# Autodesk Inventor assembly: Assembly_Cube_Lens_holder_v3
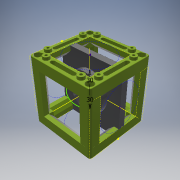
[picture p0: Inventor's stored thumbnail of the model, 180x180]
Saved by Autodesk Inventor 2019 (Build 230136000, 136)
## iProperties
Created: 2020-11-11
Part Number: Assembly_Cube_Lens_holder_v3
Document SubType Name: Assembly
Designer: marsikovabarbora
Author: marsikovabarbora
## Documents named in this file (5)
- C:\Users\UC2\Dropbox\UC2\02_CAD\INVENTOR\uc2_v3\Assembly_Cube_Lens_holder_100mm_v3.iam
- C:\Users\UC2\Dropbox\UC2\02_CAD\INVENTOR\uc2_v3\Assembly_Cube_empty_IM_v3.iam
- C:\Users\UC2\Dropbox\UC2\02_CAD\INVENTOR\uc2_v3\Imported Components\20_Insert_Lens_holder_v3\20_Insert_Lens_holder_v3_imported.ipt
- C:\Users\UC2\Dropbox\UC2\02_CAD\INVENTOR\uc2_v3\Imported Components\20_Insert_Lens_clamp_v3\20_Insert_Lens_clamp_v3.ipt
- C:\Users\UC2\Dropbox\UC2\02_CAD\INVENTOR\uc2_v3\00_Comar_Filter_25Dia.ipt
## Components (4 placed, 4 different names)
1. Assembly_Cube_empty_IM_v3:1 [sub-assembly] — Mate:1, Mate:2, Mate:3, Flush:1, Mate:7, Angle:1, Mate:8
2. 20_Insert_Lens_holder_v3_imported:1 — Mate:4, Mate:5, Mate:6, Flush:1, Angle:1
3. 20_Insert_Lens_clamp_v3_imported:1 — Mate:6, Mate:8
4. 00_Comar_Filter_25Dia:1 — Mate:4, Mate:5, Mate:7
## Relationships (10: Mate 8, Flush 1, Angle 1)
- Mate:1: Assembly_Cube_empty_IM_v3:1
- Mate:2: Assembly_Cube_empty_IM_v3:1
- Mate:3: Assembly_Cube_empty_IM_v3:1
- Mate:4: 20_Insert_Lens_holder_v3_imported:1 ↔ 00_Comar_Filter_25Dia:1
- Mate:5: 20_Insert_Lens_holder_v3_imported:1 ↔ 00_Comar_Filter_25Dia:1
- Mate:6: 20_Insert_Lens_holder_v3_imported:1 ↔ 20_Insert_Lens_clamp_v3_imported:1
- Flush:1: Assembly_Cube_empty_IM_v3:1 ↔ 20_Insert_Lens_holder_v3_imported:1
- Mate:7: Assembly_Cube_empty_IM_v3:1 ↔ 00_Comar_Filter_25Dia:1
- Angle:1 (0 deg): Assembly_Cube_empty_IM_v3:1 ↔ 20_Insert_Lens_holder_v3_imported:1
- Mate:8: Assembly_Cube_empty_IM_v3:1 ↔ 20_Insert_Lens_clamp_v3_imported:1
